# Autodesk Inventor assembly: Assembly
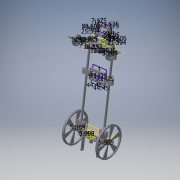
[picture p0: Inventor's stored thumbnail of the model, 180x180]
Saved by Autodesk Inventor 2018 (Build 220112000, 112)
## iProperties
Created: 2017-11-06
Part Number: Assembly
Document SubType Name: Assembly
Designer: David Cutting
Author: David Cutting
## Documents named in this file (18)
- C:\Users\Payal Jindal\Documents\Inventor\Mousetrap\Assembly.iam
- C:\Users\Payal Jindal\Documents\Inventor\Mousetrap\frontChassis_final.ipt
- C:\Users\Payal Jindal\Documents\Inventor\Mousetrap\carbonFiberTube.ipt
- C:\Users\Payal Jindal\Documents\Inventor\Mousetrap\clampCap.ipt
- C:\Users\Payal Jindal\Documents\Inventor\Mousetrap\rearChassis_final.ipt
- C:\Users\Payal Jindal\Documents\Inventor\Mousetrap\mousetrapHolder.ipt
- C:\Users\Payal Jindal\Documents\Inventor\Mousetrap\535018\bearings.ipt
- C:\Users\Payal Jindal\Documents\Inventor\Mousetrap\98873A200_MOISTURE-RESISTANT ACETAL THREADED ROD.ipt
- C:\Users\Payal Jindal\Documents\Inventor\Mousetrap\nutSecurer.ipt
- C:\Users\Payal Jindal\Documents\Inventor\Mousetrap\99223A029_ACETAL HEX NUT.ipt
- C:\Users\Payal Jindal\Documents\Inventor\Mousetrap\wheel.ipt
- C:\Users\Payal Jindal\Documents\Inventor\Mousetrap\spindleRod.ipt
- C:\Users\Payal Jindal\Documents\Inventor\Mousetrap\wheelSpindle.ipt
- C:\Users\Payal Jindal\Documents\Inventor\Mousetrap\intermediateSpindle.ipt
- C:\Users\Payal Jindal\Documents\Inventor\Mousetrap\wingnut_final.ipt
- C:\Users\Payal Jindal\Documents\Inventor\Mousetrap\washeript.ipt
- C:\Users\Payal Jindal\Documents\Inventor\Mousetrap\smallWheel.ipt
- C:\Users\Payal Jindal\Documents\Inventor\Mousetrap\springPusherAssembly.iam
## Components (50 placed, 17 different names)
1. frontChassis_final:1 — Mate:1, Mate:2, Mate:3, Mate:4, Angle:3, Flush:3, Angle:4, Flush:4, Mate:16, Mate:17, Mate:18, Mate:19, Mate:26, Angle:8
2. carbonFiberTube:1 — Mate:1, Mate:2, Mate:6, Mate:9, Mate:10, Mate:12, Mate:14
3. carbonFiberTube:2 — Mate:3, Mate:4, Mate:5, Mate:7, Mate:8, Mate:11, Mate:13, Mate:15
4. clampCap:1 — Mate:8, Angle:1, Flush:1
5. clampCap:2 — Mate:9, Angle:2, Flush:2
6. rearChassis_final:1 — Mate:5, Mate:6, Mate:7, Angle:1, Flush:1, Angle:2, Flush:2, Mate:96, Mate:97, Mate:99, Mate:109
7. clampCap:3 — Mate:10, Angle:3, Flush:3
8. clampCap:4 — Mate:11, Angle:4, Flush:4
9. mousetrapHolder:1 — Mate:12, Mate:13, Angle:5, Flush:5, Angle:6, Flush:6
10. clampCap:5 — Mate:15, Angle:6, Flush:6
11. clampCap:6 — Mate:14, Angle:5, Flush:5
12. bearings:1 — Mate:16, Mate:17, Mate:29, Mate:35
13. bearings:2 — Mate:26
14. bearings:3 — Mate:18, Mate:19, Mate:28, Mate:39
15. bearings:4 — Mate:33, Mate:98, Mate:99
16. bearings:6 — Mate:30, Mate:37, Mate:97
17. 98873A200_MOISTURE-RESISTANT ACETAL THREADED ROD:1 — Mate:30, Mate:32, Mate:36, Mate:40, Mate:42, Mate:62, Mate:64, Mate:65, Mate:76, Mate:79, Mate:80, Mate:82, Mate:93, Mate:95, Mate:96, Flush:10, Mate:98, Mate:108
18. 98873A200_MOISTURE-RESISTANT ACETAL THREADED ROD:2 — Mate:28, Mate:29, Mate:34, Mate:38, Mate:44, Mate:46, Mate:53, Mate:63, Mate:66, Mate:67, Mate:77, Mate:81, Mate:83, Mate:84, Flush:8, Mate:102, Mate:104
19. nutSecurer:1 — Mate:34, Mate:35, Mate:47
20. nutSecurer:2 — Mate:36, Mate:37, Mate:41
21. nutSecurer:3 — Mate:32, Mate:33, Mate:43
22. nutSecurer:4 — Mate:38, Mate:39, Mate:45
23. 99223A029_ACETAL HEX NUT:1 — Mate:40, Mate:41, Mate:68
24. 99223A029_ACETAL HEX NUT:2 — Mate:42, Mate:43, Mate:69
25. 99223A029_ACETAL HEX NUT:3 — Mate:46, Mate:47, Mate:70
26. 99223A029_ACETAL HEX NUT:4 — Mate:44, Mate:45, Mate:71
27. wheel:2 — Mate:104, Mate:105, Mate:106
28. wheel:4 — Mate:102, Mate:103, Mate:107
29. spindleRod:1 — Mate:54
30. wheelSpindle:1 — Mate:53, Flush:9
31. intermediateSpindle:1 — Mate:54, Flush:9
32. wingnut_final:1 — Mate:55, Mate:56, Mate:57, Mate:62, Mate:110
33. wingnut_final:2 — Mate:58, Mate:59, Mate:60, Mate:61, Mate:63, Angle:8
34. 99223A029_ACETAL HEX NUT:5 — Mate:55, Mate:56, Mate:57
35. 99223A029_ACETAL HEX NUT:6 — Mate:58, Mate:59, Mate:60, Mate:61
36. 99223A029_ACETAL HEX NUT:7 — Mate:64, Mate:68, Mate:94
37. 99223A029_ACETAL HEX NUT:8 — Mate:65, Mate:69, Mate:101
38. 99223A029_ACETAL HEX NUT:9 — Mate:67, Mate:71, Mate:107
39. 99223A029_ACETAL HEX NUT:10 — Mate:66, Mate:70, Mate:106
40. 99223A029_ACETAL HEX NUT:11 — Mate:77, Mate:91, Flush:8
41. 99223A029_ACETAL HEX NUT:12 — Mate:76, Mate:89, Flush:10
42. 99223A029_ACETAL HEX NUT:13 — Mate:79, Mate:90
43. washeript:1 — Mate:82, Mate:90, Mate:100
44. washeript:2 — Mate:81, Mate:91, Mate:103
45. washeript:4 — Mate:80, Mate:89
46. washeript:5 — Mate:83, Mate:92, Mate:105
47. 99223A029_ACETAL HEX NUT:14 — Mate:84, Mate:92
48. smallWheel:1 — Mate:95, Mate:100, Mate:101
49. smallWheel:2 — Mate:93, Mate:94
50. springPusherAssembly:3 [sub-assembly] — Mate:108, Mate:109, Mate:110
## Relationships (104: Mate 88, Flush 9, Angle 7)
- Mate:1: frontChassis_final:1 ↔ carbonFiberTube:1
- Mate:2: frontChassis_final:1 ↔ carbonFiberTube:1
- Mate:3: frontChassis_final:1 ↔ carbonFiberTube:2
- Mate:4: frontChassis_final:1 ↔ carbonFiberTube:2
- Mate:5: carbonFiberTube:2 ↔ rearChassis_final:1
- Mate:6: carbonFiberTube:1 ↔ rearChassis_final:1
- Mate:7: carbonFiberTube:2 ↔ rearChassis_final:1
- Mate:8: carbonFiberTube:2 ↔ clampCap:1
- Angle:1 (0 deg): clampCap:1 ↔ rearChassis_final:1
- Flush:1: clampCap:1 ↔ rearChassis_final:1
- Mate:9: carbonFiberTube:1 ↔ clampCap:2
- Angle:2 (0 deg): clampCap:2 ↔ rearChassis_final:1
- Flush:2: clampCap:2 ↔ rearChassis_final:1
- Mate:10: carbonFiberTube:1 ↔ clampCap:3
- Angle:3 (0 deg): frontChassis_final:1 ↔ clampCap:3
- Flush:3: frontChassis_final:1 ↔ clampCap:3
- Mate:11: carbonFiberTube:2 ↔ clampCap:4
- Angle:4 (0 deg): frontChassis_final:1 ↔ clampCap:4
- Flush:4: frontChassis_final:1 ↔ clampCap:4
- Mate:12: carbonFiberTube:1 ↔ mousetrapHolder:1
- Mate:13: carbonFiberTube:2 ↔ mousetrapHolder:1
- Mate:14: carbonFiberTube:1 ↔ clampCap:6
- Angle:5 (0 deg): mousetrapHolder:1 ↔ clampCap:6
- Flush:5: mousetrapHolder:1 ↔ clampCap:6
- Mate:15: carbonFiberTube:2 ↔ clampCap:5
- Angle:6 (0 deg): mousetrapHolder:1 ↔ clampCap:5
- Flush:6: mousetrapHolder:1 ↔ clampCap:5
- Mate:16: frontChassis_final:1 ↔ bearings:1
- Mate:17: frontChassis_final:1 ↔ bearings:1
- Mate:18: frontChassis_final:1 ↔ bearings:3
- Mate:19: frontChassis_final:1 ↔ bearings:3
- Mate:26: frontChassis_final:1 ↔ bearings:2
- Mate:28: bearings:3 ↔ 98873A200_MOISTURE-RESISTANT ACETAL THREADED ROD:2
- Mate:29: bearings:1 ↔ 98873A200_MOISTURE-RESISTANT ACETAL THREADED ROD:2
- Mate:30: bearings:6 ↔ 98873A200_MOISTURE-RESISTANT ACETAL THREADED ROD:1
- Mate:32: 98873A200_MOISTURE-RESISTANT ACETAL THREADED ROD:1 ↔ nutSecurer:3
- Mate:33: bearings:4 ↔ nutSecurer:3
- Mate:34: 98873A200_MOISTURE-RESISTANT ACETAL THREADED ROD:2 ↔ nutSecurer:1
- Mate:35: bearings:1 ↔ nutSecurer:1
- Mate:36: 98873A200_MOISTURE-RESISTANT ACETAL THREADED ROD:1 ↔ nutSecurer:2
- Mate:37: bearings:6 ↔ nutSecurer:2
- Mate:38: 98873A200_MOISTURE-RESISTANT ACETAL THREADED ROD:2 ↔ nutSecurer:4
- Mate:39: bearings:3 ↔ nutSecurer:4
- Mate:40: 98873A200_MOISTURE-RESISTANT ACETAL THREADED ROD:1 ↔ 99223A029_ACETAL HEX NUT:1
- Mate:41: nutSecurer:2 ↔ 99223A029_ACETAL HEX NUT:1
- Mate:42: 98873A200_MOISTURE-RESISTANT ACETAL THREADED ROD:1 ↔ 99223A029_ACETAL HEX NUT:2
- Mate:43: nutSecurer:3 ↔ 99223A029_ACETAL HEX NUT:2
- Mate:44: 98873A200_MOISTURE-RESISTANT ACETAL THREADED ROD:2 ↔ 99223A029_ACETAL HEX NUT:4
- Mate:45: nutSecurer:4 ↔ 99223A029_ACETAL HEX NUT:4
- Mate:46: 98873A200_MOISTURE-RESISTANT ACETAL THREADED ROD:2 ↔ 99223A029_ACETAL HEX NUT:3
- Mate:47: nutSecurer:1 ↔ 99223A029_ACETAL HEX NUT:3
- Mate:53: 98873A200_MOISTURE-RESISTANT ACETAL THREADED ROD:2 ↔ wheelSpindle:1
- Mate:54: spindleRod:1 ↔ intermediateSpindle:1
- Mate:55: wingnut_final:1 ↔ 99223A029_ACETAL HEX NUT:5
- Mate:56: wingnut_final:1 ↔ 99223A029_ACETAL HEX NUT:5
- Mate:57: wingnut_final:1 ↔ 99223A029_ACETAL HEX NUT:5
- Mate:58: wingnut_final:2 ↔ 99223A029_ACETAL HEX NUT:6
- Mate:59: wingnut_final:2 ↔ 99223A029_ACETAL HEX NUT:6
- Mate:60: wingnut_final:2 ↔ 99223A029_ACETAL HEX NUT:6
- Mate:61: wingnut_final:2 ↔ 99223A029_ACETAL HEX NUT:6
- Mate:62: 98873A200_MOISTURE-RESISTANT ACETAL THREADED ROD:1 ↔ wingnut_final:1
- Mate:63: 98873A200_MOISTURE-RESISTANT ACETAL THREADED ROD:2 ↔ wingnut_final:2
- Angle:8 (0 deg): frontChassis_final:1 ↔ wingnut_final:2
- Mate:64: 98873A200_MOISTURE-RESISTANT ACETAL THREADED ROD:1 ↔ 99223A029_ACETAL HEX NUT:7
- Mate:65: 98873A200_MOISTURE-RESISTANT ACETAL THREADED ROD:1 ↔ 99223A029_ACETAL HEX NUT:8
- Mate:66: 98873A200_MOISTURE-RESISTANT ACETAL THREADED ROD:2 ↔ 99223A029_ACETAL HEX NUT:10
- Mate:67: 98873A200_MOISTURE-RESISTANT ACETAL THREADED ROD:2 ↔ 99223A029_ACETAL HEX NUT:9
- Mate:68: 99223A029_ACETAL HEX NUT:1 ↔ 99223A029_ACETAL HEX NUT:7
- Mate:69: 99223A029_ACETAL HEX NUT:2 ↔ 99223A029_ACETAL HEX NUT:8
- Mate:70: 99223A029_ACETAL HEX NUT:3 ↔ 99223A029_ACETAL HEX NUT:10
- Mate:71: 99223A029_ACETAL HEX NUT:4 ↔ 99223A029_ACETAL HEX NUT:9
- Mate:76: 98873A200_MOISTURE-RESISTANT ACETAL THREADED ROD:1 ↔ 99223A029_ACETAL HEX NUT:12
- Mate:77: 98873A200_MOISTURE-RESISTANT ACETAL THREADED ROD:2 ↔ 99223A029_ACETAL HEX NUT:11
- Mate:79: 98873A200_MOISTURE-RESISTANT ACETAL THREADED ROD:1 ↔ 99223A029_ACETAL HEX NUT:13
- Mate:80: 98873A200_MOISTURE-RESISTANT ACETAL THREADED ROD:1 ↔ washeript:4
- Mate:81: 98873A200_MOISTURE-RESISTANT ACETAL THREADED ROD:2 ↔ washeript:2
- Mate:82: 98873A200_MOISTURE-RESISTANT ACETAL THREADED ROD:1 ↔ washeript:1
- Mate:83: 98873A200_MOISTURE-RESISTANT ACETAL THREADED ROD:2 ↔ washeript:5
- Mate:84: 98873A200_MOISTURE-RESISTANT ACETAL THREADED ROD:2 ↔ 99223A029_ACETAL HEX NUT:14
- Mate:89: 99223A029_ACETAL HEX NUT:12 ↔ washeript:4
- Mate:90: 99223A029_ACETAL HEX NUT:13 ↔ washeript:1
- Mate:91: 99223A029_ACETAL HEX NUT:11 ↔ washeript:2
- Mate:92: washeript:5 ↔ 99223A029_ACETAL HEX NUT:14
- Flush:8: 98873A200_MOISTURE-RESISTANT ACETAL THREADED ROD:2 ↔ 99223A029_ACETAL HEX NUT:11
- Flush:9: wheelSpindle:1 ↔ intermediateSpindle:1
- Mate:93: 98873A200_MOISTURE-RESISTANT ACETAL THREADED ROD:1 ↔ smallWheel:2
- Mate:94: 99223A029_ACETAL HEX NUT:7 ↔ smallWheel:2
- Mate:95: 98873A200_MOISTURE-RESISTANT ACETAL THREADED ROD:1 ↔ smallWheel:1
- Mate:96: rearChassis_final:1 ↔ 98873A200_MOISTURE-RESISTANT ACETAL THREADED ROD:1
- Mate:97: rearChassis_final:1 ↔ bearings:6
- Flush:10: 98873A200_MOISTURE-RESISTANT ACETAL THREADED ROD:1 ↔ 99223A029_ACETAL HEX NUT:12
- Mate:98: bearings:4 ↔ 98873A200_MOISTURE-RESISTANT ACETAL THREADED ROD:1
- Mate:99: rearChassis_final:1 ↔ bearings:4
- Mate:100: washeript:1 ↔ smallWheel:1
- Mate:101: 99223A029_ACETAL HEX NUT:8 ↔ smallWheel:1
- Mate:102: 98873A200_MOISTURE-RESISTANT ACETAL THREADED ROD:2 ↔ wheel:4
- Mate:103: wheel:4 ↔ washeript:2
- Mate:104: 98873A200_MOISTURE-RESISTANT ACETAL THREADED ROD:2 ↔ wheel:2
- Mate:105: wheel:2 ↔ washeript:5
- Mate:106: wheel:2 ↔ 99223A029_ACETAL HEX NUT:10
- Mate:107: wheel:4 ↔ 99223A029_ACETAL HEX NUT:9
- Mate:108: 98873A200_MOISTURE-RESISTANT ACETAL THREADED ROD:1 ↔ springPusherAssembly:3
- Mate:109: rearChassis_final:1 ↔ springPusherAssembly:3
- Mate:110: wingnut_final:1 ↔ springPusherAssembly:3
